# Autodesk Inventor assembly: Assembly1
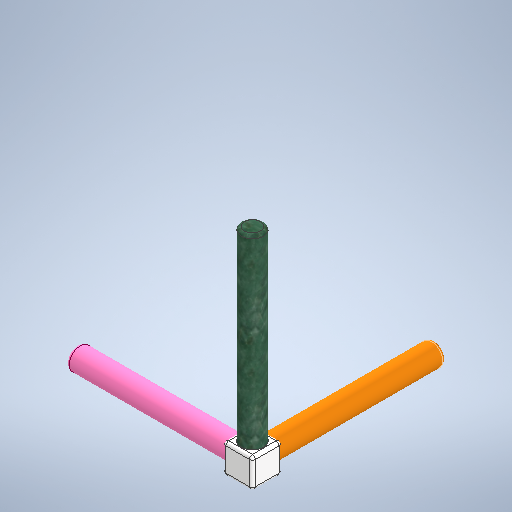
[picture p0: Inventor's stored thumbnail of the model, 512x512]
Saved by Autodesk Inventor 2025 (Build 290162000, 162)
## iProperties
Created: 2026-02-12
Part Number: Assembly1
Document SubType Name: Assembly
Designer: tapen
Author: tapen
## Documents named in this file (3)
- C:\Users\tapen\OneDrive\Desktop\Vesna Milosevic-Zdjelar\3Axis\Assembly1.iam
- C:\Users\tapen\OneDrive\Desktop\Vesna Milosevic-Zdjelar\3Axis\Center.ipt
- C:\Users\tapen\OneDrive\Desktop\Vesna Milosevic-Zdjelar\3Axis\axis.ipt
## Components (4 placed, 2 different names)
1. Center:1 — Mate:1, Mate:2, Mate:3
2. axis:1 — Mate:3
3. axis:2 — Mate:1
4. axis:3 — Mate:2
## Relationships (3: Mate 3)
- Mate:1: Center:1 ↔ axis:2
- Mate:2: Center:1 ↔ axis:3
- Mate:3: Center:1 ↔ axis:1
